# Autodesk Inventor assembly: Frame 1609825998716
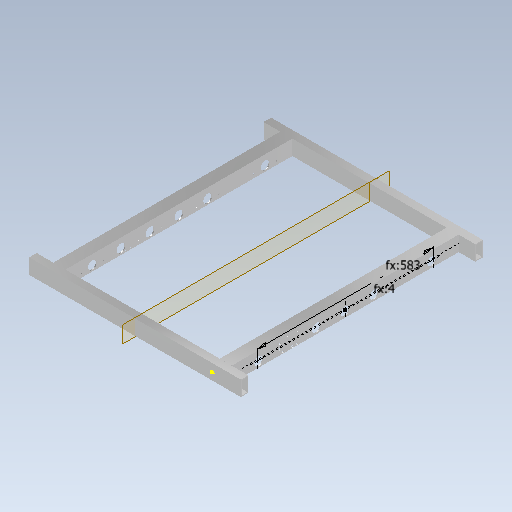
[picture p0: Inventor's stored thumbnail of the model, 512x512]
Saved by Autodesk Inventor 2021 (Build 250183000, 183)
## iProperties
_FrameDoc: Frame Assembly
_Version: 25.0.0
Created: 2021-01-05
Part Number: Frame 1609825998716
Document SubType Name: Assembly
Designer: lucky
Mass: 3107.99 g
Surface Area: 7889.54 cm^2
Volume: 1151.11 cm^3
Density: 2.7 g/cm^3
Author: lucky
## Documents named in this file (8)
- C:\Users\lucky\Documents\Inventor\2020DRIVEBASE\Frame 1609825998716.iam
- WCD CHASSI.iam
- C:\Users\lucky\Documents\Inventor\2020DRIVEBASE\CHASSI SIDE PIECES.ipt
- C:\Users\lucky\Documents\Inventor\2020DRIVEBASE\1609907106059.ipt
- C:\Users\lucky\Documents\Inventor\2020DRIVEBASE\1609907106065.ipt
- C:\Users\lucky\Documents\Inventor\2020DRIVEBASE\1609907106067.ipt
- C:\Users\lucky\Documents\Inventor\2020DRIVEBASE\1609907106069.ipt
- C:\Users\lucky\Documents\Inventor\2020DRIVEBASE\FRC 2021\WCD2021.xlsx
## Components (5 placed, 5 different names)
1. Frame Reference Model
2. WCD FRONT:1
3. WCD SIDE RIGHT:2 — Symmetry:1
4. WCD SIDE LEFT:3 — Symmetry:1
5. WCD BACK:4 — Flush:1
## Relationships (2: Flush 1, Symmetry 1)
- Flush:1 (-350 mm): WCD BACK:4
- Symmetry:1: WCD SIDE RIGHT:2 ↔ WCD SIDE LEFT:3
## Named parameters: Chassi_Length = 800 mm, Chassi_Width = 700 mm, Chassi_CentreDrop = 4 mm, WheelBay_Depth = 55 mm, Wheel_Qty = 3, Wheel_Diametre = 152.4 mm, Wheel_Seperation = 285.75 mm, Wheel_HightOffset = 2 mm, Wheel_Clearance = 13.05 mm, RHS_Width = 40 mm, RHS_Height = 50 mm, Wheel_HeightOffset = 4 mm, Chassi_GroundClearance = 10.116 mm, Wheel_CentreDrop = 4 mm, Wheel_Seperation2 = 194.33333 mm, Wheel_Diametre2 = 101.6 mm, Wheel_HeightOffset2 = 4 mm, Wheel_Qty2 = 4, Wheel_Clearance2 = 32.7 mm, Chain_Pitch = 9.525 mm, Wheel_MaxSeperation = 285.75 mm, Sprocket_Teeth = 12, Wheel_CCSpan = 571.5 mm, Wheel_CCSpan2 = 471.5 mm, Wheel_MaxSeperation2 = 190.5 mm, MotorholeCC = 95.25 mm, MotorholeHorizontal = 95.01318 mm, OutputshaftTopOffset = 30.058 mm, Heightfromcenter = 6.7125 mm, Chassi_SideRivetAmt = 4, Chassi_SideRivetSpacing = 37.5 mm, Sprocket_Thickness = 10.668 mm, BumperMountingBarOffset = 177.8 mm
